# Autodesk Inventor assembly: baseCapAnd2020Threads
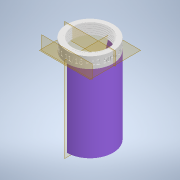
[picture p0: Inventor's stored thumbnail of the model, 180x180]
Saved by Autodesk Inventor 2021.1 (Build 251245010, 245A)
## iProperties
Created: 2020-10-12
Part Number: baseCapAnd2020Threads
Document SubType Name: Assembly
Designer: robst
Author: robst
## Documents named in this file (3)
- C:\git\CAD-Development\robSteele\ShapeWays\TelescopeProjects\eyepieceCases\baseCapAnd2020Threads.iam
- C:\git\CAD-Development\robSteele\ShapeWays\TelescopeProjects\eyepieceCases\BaseForSvBonyPlosse-40mm.ipt
- C:\git\CAD-Development\robSteele\ShapeWays\TelescopeProjects\eyepieceCases\2020-threadsForBody.ipt
## Components (2 placed, 2 different names)
1. BaseForSvBonyPlosse-40mm:1 — Insert:1
2. 2020-threadsForBody:1 — Insert:1
## Relationships (1: Insert 1)
- Insert:1: BaseForSvBonyPlosse-40mm:1 ↔ 2020-threadsForBody:1
